# Autodesk Inventor assembly: Assembly1
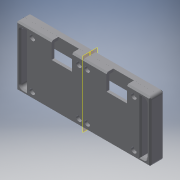
[picture p0: Inventor's stored thumbnail of the model, 180x180]
Saved by Autodesk Inventor 2017 (Build 210142000, 142)
## iProperties
Created: 2017-04-10
Part Number: Assembly1
Document SubType Name: Assembly
Designer: Matt Bierner
Author: Matt Bierner
## Documents named in this file (3)
- C:\Users\Matt Bierner\SkyDrive\projects\camera-housing-stereo\Assembly1.iam
- C:\Users\Matt Bierner\SkyDrive\projects\camera-housing-stereo\back-stereo.ipt
- C:\Users\Matt Bierner\SkyDrive\projects\camera-housing-stereo\front-stereo.ipt
## Components (2 placed, 2 different names)
1. back-stereo:1 — Mate:1, Mate:2, Mate:3
2. front-stereo:1 — Mate:1, Mate:2, Mate:3
## Relationships (3: Mate 3)
- Mate:1: back-stereo:1 ↔ front-stereo:1
- Mate:2: back-stereo:1 ↔ front-stereo:1
- Mate:3: back-stereo:1 ↔ front-stereo:1
